# Autodesk Inventor assembly: 217-2709-101 Rev1
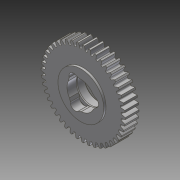
[picture p0: Inventor's stored thumbnail of the model, 180x180]
Saved by Autodesk Inventor 2014 SP1 (Build 180222100, 222)
## iProperties
Created: 2014-01-07
Part Number: 217-2709-101 Rev1
Document SubType Name: Assembly
Designer: Andrew Toennies
Mass: 167.777 g
Surface Area: 100.733 cm^2
Volume: 21.3729 cm^3
Density: 7.85 g/cm^3
Author: Andrew Toennies
## Documents named in this file (3)
- C:\Users\Moses\Documents\Inventor\Robot\Constrained 2 Speed Ball Shifter\217-2709-101 Rev1.iam
- C:\Users\Moses\Documents\Inventor\Robot\Constrained 2 Speed Ball Shifter\217-2428-022 Rev1.ipt
- C:\Users\Moses\Documents\Inventor\Robot\Constrained 2 Speed Ball Shifter\217-2709-001_44t Steel.ipt
## Components (2 placed, 2 different names)
1. 217-2428-022 Rev1_71 — Insert:1
2. 217-2709-001_44t Steel_72 — Insert:1
## Relationships (1: Insert 1)
- Insert:1: 217-2428-022 Rev1_71 ↔ 217-2709-001_44t Steel_72
